# Autodesk Inventor assembly: leftarm
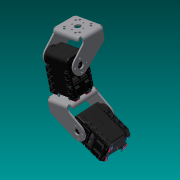
[picture p0: Inventor's stored thumbnail of the model, 180x180]
Saved by Autodesk Inventor 2013 SP2 (Build 170200200, 200)
## iProperties
Created: 2014-11-26
Part Number: leftarm
Document SubType Name: Assembly
Designer: Master
Author: Master
## Documents named in this file (3)
- C:\Users\Master\Documents\GitHub\DIY-HR-OS1\CAD Files\leftarm.iam
- C:\Users\Master\Documents\GitHub\DIY-HR-OS1\CAD Files\45angle.ipt
- C:\Users\Master\Documents\GitHub\DIY-HR-OS1\CAD Files\AX12\AX12.iam
## Components (4 placed, 2 different names)
1. 45angle:1 — Mate:1, Mate:2, Mate:6
2. AX12:1 [sub-assembly] — Mate:1, Mate:2, Mate:3, Mate:4, Mate:5
3. 45angle:2 — Mate:3, Mate:4, Mate:5, Mate:7, Mate:8
4. AX12:2 [sub-assembly] — Mate:7, Mate:8
## Relationships (8: Mate 8)
- Mate:1: 45angle:1 ↔ AX12:1
- Mate:2: 45angle:1 ↔ AX12:1
- Mate:3: AX12:1 ↔ 45angle:2
- Mate:4: AX12:1 ↔ 45angle:2
- Mate:5: AX12:1 ↔ 45angle:2
- Mate:6: 45angle:1
- Mate:7: 45angle:2 ↔ AX12:2
- Mate:8: 45angle:2 ↔ AX12:2
